# Autodesk Inventor assembly: PA_0001_001
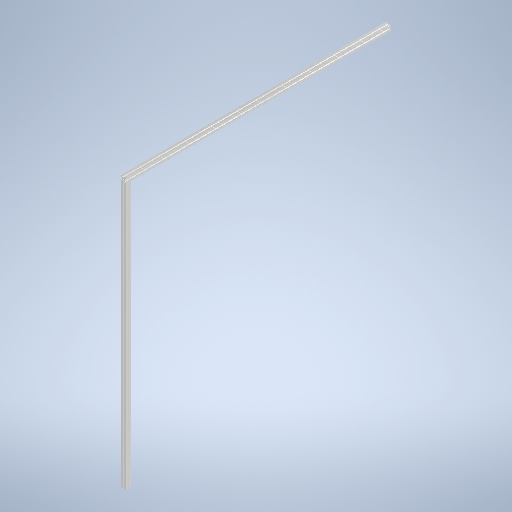
[picture p0: Inventor's stored thumbnail of the model, 512x512]
Saved by Autodesk Inventor 2026 (Build 300175000, 175)
## iProperties
Created: 2025-03-28
Part Number: PA_0001_001
Document SubType Name: Assembly
Designer: Carlos Dias
Author: Carlos Dias
## Documents named in this file (3)
- C:\Users\Carlos Dias\Documents\Formação-TEARCI\UFCDs\5134 - Robótica _ Fundamentos\Material De Apoio\Sessao_25_03\PA_0001_001.iam
- C:\Users\Carlos Dias\Documents\Formação-TEARCI\UFCDs\5134 - Robótica _ Fundamentos\Material De Apoio\Sessao_25_03\perfil_20x20_001.ipt
- C:\Users\Carlos Dias\Documents\Formação-TEARCI\UFCDs\5134 - Robótica _ Fundamentos\Material De Apoio\Sessao_25_03\perfil_20x20_002.ipt
## Components (2 placed, 2 different names)
1. perfil_20x20_001:1 — Flush:1, Flush:2, Flush:3, Mate:1, Flush:4
2. perfil_20x20_002:1 — Mate:1, Flush:4, Mate:2
## Relationships (6: Flush 4, Mate 2)
- Flush:1: perfil_20x20_001:1
- Flush:2: perfil_20x20_001:1
- Flush:3: perfil_20x20_001:1
- Mate:1: perfil_20x20_001:1 ↔ perfil_20x20_002:1
- Flush:4: perfil_20x20_001:1 ↔ perfil_20x20_002:1
- Mate:2 (490 mm): perfil_20x20_002:1
